# Autodesk Inventor assembly: MicAssembly
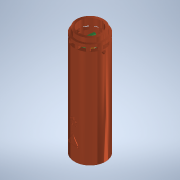
[picture p0: Inventor's stored thumbnail of the model, 180x180]
Saved by Autodesk Inventor 2020 (Build 240168000, 168)
## iProperties
Created: 2020-06-09
Part Number: MicAssembly
Document SubType Name: Assembly
Designer: vmiguel
Author: vmiguel
## Documents named in this file (6)
- C:\Github\Wintergatan-MMX-Microphone\CAD\MicAssembly.iam
- C:\Github\Wintergatan-MMX-Microphone\CAD\CapsuleBody.ipt
- C:\Github\Wintergatan-MMX-Microphone\CAD\PreAmpBody.ipt
- C:\Github\Wintergatan-MMX-Microphone\CAD\CapuleScreen.ipt
- C:\Github\Wintergatan-MMX-Microphone\CAD\NeutrikXLR.ipt
- C:\Github\Wintergatan-MMX-Microphone\PCB\MicAmp_Final.ipt
## Components (5 placed, 5 different names)
1. CapsuleBody:1 — Mate:8, Mate:9, Rotational:1
2. PreAmpBody:1 — Mate:10, Rotational:1, Mate:14, Angle:1
3. CapuleScreen:1 — Mate:8, Mate:9
4. NeutrikXLR:1 — Mate:10, Mate:11, Mate:13, Angle:1, Angle:2, Mate:15
5. MicAmp_Final:1 — Mate:11, Mate:13, Mate:14, Angle:2, Mate:15
## Relationships (10: Mate 7, Angle 2, RevoluteJoint 1)
- Mate:8: CapsuleBody:1 ↔ CapuleScreen:1
- Mate:9: CapsuleBody:1 ↔ CapuleScreen:1
- Mate:10: PreAmpBody:1 ↔ NeutrikXLR:1
- Rotational:1 [RevoluteJoint]: CapsuleBody:1 ↔ PreAmpBody:1
- Mate:11: NeutrikXLR:1 ↔ MicAmp_Final:1
- Mate:13: NeutrikXLR:1 ↔ MicAmp_Final:1
- Mate:14: PreAmpBody:1 ↔ MicAmp_Final:1
- Angle:1 (135 deg): PreAmpBody:1 ↔ NeutrikXLR:1
- Angle:2 (0 deg): NeutrikXLR:1 ↔ MicAmp_Final:1
- Mate:15: NeutrikXLR:1 ↔ MicAmp_Final:1
